# Autodesk Inventor assembly: POM_T5_27
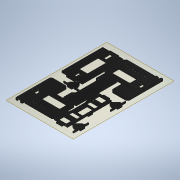
[picture p0: Inventor's stored thumbnail of the model, 180x180]
Saved by Autodesk Inventor 2020 (Build 240168000, 168)
## iProperties
Created: 2021-08-27
Part Number: POM_T5_27
Document SubType Name: Assembly
Designer: Masato
Author: Masato
## Documents named in this file (7)
- C:\Inventor\SUSTAINA-OP\Cam\POM_T5_27.iam
- C:\Inventor\SUSTAINA-OP\Cam\DisposableBoard.ipt
- C:\Inventor\SUSTAINA-OP\UpperBody\Cockpit\Cockpit_battery_back_door.ipt
- C:\Inventor\SUSTAINA-OP\UpperBody\Cockpit\Cockpit_side_frame.ipt
- C:\Inventor\SUSTAINA-OP\UpperBody\Cockpit\Cockpit_back_frame.ipt
- C:\Inventor\SUSTAINA-OP\UpperBody\Trunk\Trunk_chest_frame.ipt
- C:\Inventor\SUSTAINA-OP\UpperBody\Head\Camera_side_frame.ipt
## Components (9 placed, 6 different names)
1. DisposableBoard:1 — メイト:2, メイト:1, フラッシュ:1, フラッシュ:2, メイト:4, フラッシュ:3, フラッシュ:4, メイト:5, メイト:6, メイト:7, メイト:8, メイト:12, メイト:13
2. Cockpit_side_frame:1 — メイト:4, フラッシュ:3, フラッシュ:4, メイト:9, フラッシュ:5, メイト:10, メイト:14, フラッシュ:6
3. Cockpit_back_frame:1 — メイト:5, 正接:1, フラッシュ:6, メイト:17
4. Trunk_chest_frame:1 — メイト:6, フラッシュ:5, メイト:10, メイト:11, フラッシュ:7, 正接:2
5. Cockpit_battery_back_door:1 — メイト:7, メイト:9, メイト:11, メイト:15, メイト:16
6. Cockpit_side_frame:2 — メイト:8, メイト:16, メイト:17
7. Camera_side_frame:1 — メイト:12, メイト:14, メイト:15, 正接:1
8. Camera_side_frame:2 — メイト:13, フラッシュ:7, 正接:2
9. Camera_side_frame:3
## Component patterns: (2 elements, first: Camera_side_frame:2)
## Relationships (25: Mate 16, Flush 7, Tangent 2)
- メイト:2 [Mate]: DisposableBoard:1
- メイト:1 [Mate]: DisposableBoard:1
- フラッシュ:1 [Flush]: DisposableBoard:1
- フラッシュ:2 [Flush]: DisposableBoard:1
- メイト:4 [Mate]: DisposableBoard:1 ↔ Cockpit_side_frame:1
- フラッシュ:3 [Flush] (2 mm): DisposableBoard:1 ↔ Cockpit_side_frame:1
- フラッシュ:4 [Flush] (2 mm): DisposableBoard:1 ↔ Cockpit_side_frame:1
- メイト:5 [Mate]: DisposableBoard:1 ↔ Cockpit_back_frame:1
- メイト:6 [Mate]: DisposableBoard:1 ↔ Trunk_chest_frame:1
- メイト:7 [Mate]: DisposableBoard:1 ↔ Cockpit_battery_back_door:1
- メイト:8 [Mate]: DisposableBoard:1 ↔ Cockpit_side_frame:2
- メイト:9 [Mate] (2.5 mm): Cockpit_side_frame:1 ↔ Cockpit_battery_back_door:1
- フラッシュ:5 [Flush]: Cockpit_side_frame:1 ↔ Trunk_chest_frame:1
- メイト:10 [Mate] (2.1 mm): Cockpit_side_frame:1 ↔ Trunk_chest_frame:1
- メイト:11 [Mate] (2.5 mm): Trunk_chest_frame:1 ↔ Cockpit_battery_back_door:1
- メイト:12 [Mate]: DisposableBoard:1 ↔ Camera_side_frame:1
- メイト:13 [Mate]: DisposableBoard:1 ↔ Camera_side_frame:2
- メイト:14 [Mate] (2.5 mm): Cockpit_side_frame:1 ↔ Camera_side_frame:1
- メイト:15 [Mate] (2.5 mm): Cockpit_battery_back_door:1 ↔ Camera_side_frame:1
- 正接:1 [Tangent] (2.5 mm): Cockpit_back_frame:1 ↔ Camera_side_frame:1
- フラッシュ:6 [Flush]: Cockpit_side_frame:1 ↔ Cockpit_back_frame:1
- フラッシュ:7 [Flush]: Trunk_chest_frame:1 ↔ Camera_side_frame:2
- 正接:2 [Tangent] (2.1 mm): Trunk_chest_frame:1 ↔ Camera_side_frame:2
- メイト:16 [Mate] (2.5 mm): Cockpit_battery_back_door:1 ↔ Cockpit_side_frame:2
- メイト:17 [Mate] (2.5 mm): Cockpit_back_frame:1 ↔ Cockpit_side_frame:2
